# Autodesk Inventor assembly: HbFinger01
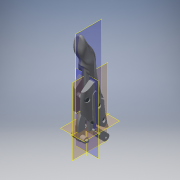
[picture p0: Inventor's stored thumbnail of the model, 180x180]
Saved by Autodesk Inventor 2016 (Build 200138000, 138)
## iProperties
Created: 2015-04-11
Part Number: HbFinger01
Document SubType Name: Assembly
Designer: Yamaura
Author: Yamaura
## Documents named in this file (8)
- C:\Users\Yamaura\Documents\GitHub\HACKberry\HACKberry-hardware\3D\Inventor\Parts\HbFinger01.iam
- C:\Users\Yamaura\Documents\GitHub\HACKberry\HACKberry-hardware\3D\Inventor\Parts\HbFingerPosture02.ipt
- C:\Users\Yamaura\Documents\GitHub\HACKberry\HACKberry-hardware\3D\Inventor\Parts\HbMiddle-DistalPhalanx02.ipt
- C:\Users\Yamaura\Documents\GitHub\HACKberry\HACKberry-hardware\3D\Inventor\Parts\HbProximalPhalanx02.ipt
- C:\Users\Yamaura\Documents\GitHub\HACKberry\HACKberry-hardware\3D\Inventor\Parts\HbProximalPhalanxCover02.ipt
- C:\Users\Yamaura\Documents\GitHub\HACKberry\HACKberry-hardware\3D\Inventor\Parts\HbCouplerLink02.ipt
- C:\Users\Yamaura\Documents\GitHub\HACKberry\HACKberry-hardware\3D\Inventor\Parts\HbCouplerLinkCover03.ipt
- C:\Users\Yamaura\Documents\GitHub\HACKberry\HACKberry-hardware\3D\Inventor\Parts\ScrewM2L10.ipt
## Components (10 placed, 7 different names)
1. HbFingerPosture01_1
2. HbMiddle-DistalPhalanx02_1
3. HbProximalPhalanx02_1
4. HbProximalPhalanxCover02_1 — メイト:1, メイト:3, フラッシュ:1, メイト:7
5. HbCouplerLink02_1 — メイト:2, メイト:4, メイト:5, メイト:6
6. HbCouplerLinkCover03_1
7. ScrewM2L10:1 — メイト:1, フラッシュ:1
8. ScrewM2L10:2 — メイト:2, メイト:5
9. ScrewM2L10:3 — メイト:3, メイト:7
10. ScrewM2L10:4 — メイト:4, メイト:6
## Relationships (8: Mate 7, Flush 1)
- メイト:1 [Mate]: HbProximalPhalanxCover02_1 ↔ ScrewM2L10:1
- メイト:2 [Mate]: HbCouplerLink02_1 ↔ ScrewM2L10:2
- メイト:3 [Mate]: HbProximalPhalanxCover02_1 ↔ ScrewM2L10:3
- メイト:4 [Mate]: HbCouplerLink02_1 ↔ ScrewM2L10:4
- フラッシュ:1 [Flush] (2.5 mm): HbProximalPhalanxCover02_1 ↔ ScrewM2L10:1
- メイト:5 [Mate]: HbCouplerLink02_1 ↔ ScrewM2L10:2
- メイト:6 [Mate]: HbCouplerLink02_1 ↔ ScrewM2L10:4
- メイト:7 [Mate] (-1 mm): HbProximalPhalanxCover02_1 ↔ ScrewM2L10:3
